# Autodesk Inventor assembly: 207
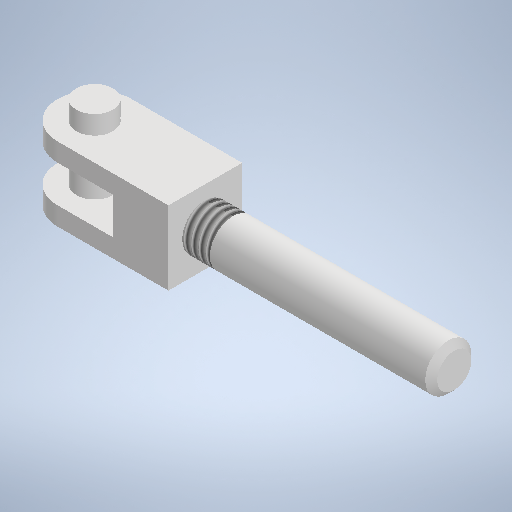
[picture p0: Inventor's stored thumbnail of the model, 512x512]
Saved by Autodesk Inventor 2025.1 (Build 291241000, 241)
## iProperties
Created: 2024-08-23
Part Number: 207
Document SubType Name: Assembly
Designer: ffogue
Author: ffogue
## Documents named in this file (4)
- C:\Projkete - Übungen\Freedom\207.iam
- C:\Projkete - Übungen\Freedom\207 part 2.ipt
- C:\Projkete - Übungen\Freedom\207 part 1.ipt
- C:\Projkete - Übungen\Freedom\207 part 3.ipt
## Components (3 placed, 3 different names)
1. 207 part 2:1 — Mate:1, Flush:1, Mate:2, Flush:2
2. 207 part 1:1 — Mate:1, Flush:1
3. 207 part 3:1 — Mate:2, Flush:2
## Relationships (4: Mate 2, Flush 2)
- Mate:1: 207 part 2:1 ↔ 207 part 1:1
- Flush:1: 207 part 2:1 ↔ 207 part 1:1
- Mate:2: 207 part 2:1 ↔ 207 part 3:1
- Flush:2 (-2 mm): 207 part 2:1 ↔ 207 part 3:1
